# Autodesk Inventor assembly: TR1 Actuator
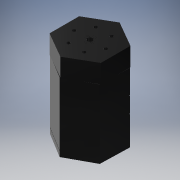
[picture p0: Inventor's stored thumbnail of the model, 180x180]
Saved by Autodesk Inventor 2017 (Build 210142000, 142)
## iProperties
Created: 2018-10-09
Part Number: TR1 Actuator
Document SubType Name: Assembly
Designer: Zach
Author: Zach
## Documents named in this file (8)
- C:\Users\Dell\Documents\GitHub\tr2\Arm Actuator\Arm Actuator.iam
- C:\Users\Dell\Documents\GitHub\tr2\Arm Actuator\TA01.ipt
- C:\Users\Dell\Documents\GitHub\tr2\Arm Actuator\TA02.ipt
- C:\Users\Dell\Documents\GitHub\tr2\Arm Actuator\Arm Actuator\Design Accelerator\Spur Gears2.iam
- C:\Users\Dell\Documents\GitHub\tr2\Arm Actuator\Arm Actuator\Design Accelerator\Spur Gears3.iam
- C:\Users\Dell\Documents\GitHub\tr2\Arm Actuator\TA03.ipt
- C:\Users\Dell\Documents\GitHub\tr2\Arm Actuator\EMS22XXX-D28-LSX.ipt
- C:\Users\Dell\Documents\GitHub\tr2\Arm Actuator\12RPM Gear Motor.ipt
## Components (10 placed, 6 different names)
1. TA01:1 — Mate:28, Mate:29, Mate:30
2. TA02:1 — Mate:2, Mate:3, Mate:4, Mate:5, Mate:6, Mate:7, Mate:8, Mate:16, Mate:17, Mate:18, Mate:19, Angle:1, Angle:2, Mate:20, Mate:21, Mate:22, Mate:24, Mate:28, Mate:29, Mate:30
3. Spur Gears:1 [sub-assembly] — Mate:2, Mate:25, Mate:26
4. Spur Gears:2 [sub-assembly] — Mate:3, Mate:4
5. Spur Gears:3 [sub-assembly] — Mate:5, Mate:6
6. TA03:1 — Mate:7, Mate:8, Mate:25, Mate:26
7. EMS22XXX-D28-LSX:1 — Mate:16, Mate:19, Angle:1, Mate:23
8. EMS22XXX-D28-LSX:2 — Mate:17, Mate:18, Angle:2
9. 12RPM Gear Motor:1 — Mate:20, Mate:21, Mate:22
10. Spur Gears:4 [sub-assembly] — Mate:23, Mate:24
## Relationships (23: Mate 21, Angle 2)
- Mate:2: TA02:1 ↔ Spur Gears:1
- Mate:3: TA02:1 ↔ Spur Gears:2
- Mate:4: TA02:1 ↔ Spur Gears:2
- Mate:5: TA02:1 ↔ Spur Gears:3
- Mate:6: TA02:1 ↔ Spur Gears:3
- Mate:7: TA02:1 ↔ TA03:1
- Mate:8: TA02:1 ↔ TA03:1
- Mate:16: TA02:1 ↔ EMS22XXX-D28-LSX:1
- Mate:17: TA02:1 ↔ EMS22XXX-D28-LSX:2
- Mate:18: TA02:1 ↔ EMS22XXX-D28-LSX:2
- Mate:19: TA02:1 ↔ EMS22XXX-D28-LSX:1
- Angle:1 (0 deg): TA02:1 ↔ EMS22XXX-D28-LSX:1
- Angle:2 (0 deg): TA02:1 ↔ EMS22XXX-D28-LSX:2
- Mate:20: TA02:1 ↔ 12RPM Gear Motor:1
- Mate:21: TA02:1 ↔ 12RPM Gear Motor:1
- Mate:22: TA02:1 ↔ 12RPM Gear Motor:1
- Mate:23: EMS22XXX-D28-LSX:1 ↔ Spur Gears:4
- Mate:24: TA02:1 ↔ Spur Gears:4
- Mate:25: Spur Gears:1 ↔ TA03:1
- Mate:26: Spur Gears:1 ↔ TA03:1
- Mate:28: TA01:1 ↔ TA02:1
- Mate:29: TA01:1 ↔ TA02:1
- Mate:30: TA01:1 ↔ TA02:1
